# Autodesk Inventor assembly: board_ver2
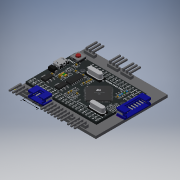
[picture p0: Inventor's stored thumbnail of the model, 180x180]
Saved by Autodesk Inventor 2019 (Build 230136000, 136)
## iProperties
Created: 2020-03-31
Part Number: board_ver2
Document SubType Name: Assembly
Designer: Pulag
Author: Pulag
## Documents named in this file (7)
- C:\Users\Pulag\Documents\GitHub\24th_TDK_Project_D5\CAD\frame\board_ver2.iam
- C:\Users\Pulag\Documents\GitHub\24th_TDK_Project_D5\CAD\frame\board_v2.ipt
- C:\Users\Pulag\Documents\GitHub\24th_TDK_Project_D5\CAD\Syno_borad_3D\匯出\B4B-PH-SM4-TB.ipt
- C:\Users\Pulag\Documents\GitHub\24th_TDK_Project_D5\CAD\Syno_borad_3D\匯出\B8B-PH-SM4-TB.ipt
- C:\Users\Pulag\Documents\GitHub\24th_TDK_Project_D5\CAD\CAD file\MEGA 2560 PRO (EMBED).iam
- C:\Users\Pulag\Documents\GitHub\24th_TDK_Project_D5\CAD\frame\geo.ipt
- C:\Users\Pulag\Documents\GitHub\24th_TDK_Project_D5\CAD\frame\measure.ipt
## Components (6 placed, 6 different names)
1. board_v2:1 — Mate:1, Flush:1, Mate:4, Mate:7, Flush:2, Flush:3, Flush:4
2. B4B-PH-SM4-TB:1 — Mate:1, Mate:2, Mate:3
3. B8B-PH-SM4-TB:1 — Mate:4, Angle:1, Mate:5, Mate:6
4. MEGA 2560 PRO (EMBED):1 [sub-assembly] — Angle:2, Mate:7, Flush:2, Flush:3
5. geo:1 — Flush:1, Mate:2, Mate:3, Angle:1, Mate:5, Mate:6, Angle:2
6. measure:1 — Flush:4
## Relationships (13: Mate 7, Flush 4, Angle 2)
- Mate:1: board_v2:1 ↔ B4B-PH-SM4-TB:1
- Flush:1: board_v2:1 ↔ geo:1
- Mate:2: B4B-PH-SM4-TB:1 ↔ geo:1
- Mate:3: B4B-PH-SM4-TB:1 ↔ geo:1
- Mate:4: board_v2:1 ↔ B8B-PH-SM4-TB:1
- Angle:1 (180 deg): B8B-PH-SM4-TB:1 ↔ geo:1
- Mate:5: B8B-PH-SM4-TB:1 ↔ geo:1
- Mate:6: B8B-PH-SM4-TB:1 ↔ geo:1
- Angle:2 (0 deg): MEGA 2560 PRO (EMBED):1 ↔ geo:1
- Mate:7: board_v2:1 ↔ MEGA 2560 PRO (EMBED):1
- Flush:2 (0.762 mm): board_v2:1 ↔ MEGA 2560 PRO (EMBED):1
- Flush:3 (7.62 mm): board_v2:1 ↔ MEGA 2560 PRO (EMBED):1
- Flush:4: board_v2:1 ↔ measure:1
